# Autodesk Inventor assembly: LearningKitSolarAlt
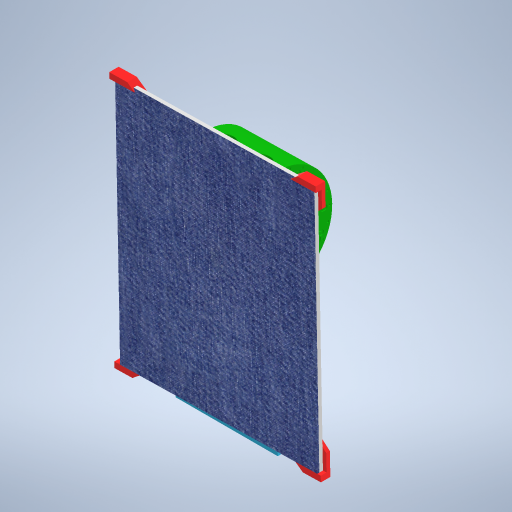
[picture p0: Inventor's stored thumbnail of the model, 512x512]
Saved by Autodesk Inventor 2024.3 (Build 283343000, 343)
## iProperties
Created: 2025-02-03
Part Number: LearningKitSolarAlt
Document SubType Name: Assembly
Designer: Maximilian Hock
Author: Maximilian Hock
## Documents named in this file (6)
- Z:\Dokumente\LearningKit\LearningKitSolar\LearningKitSolar.iam
- Z:\Dokumente\LearningKit\LearningKitSolar\SolarCradle.ipt
- Z:\Dokumente\LearningKit\LearningKitSolar\SolarFoot.ipt
- Z:\Dokumente\LearningKit\LearningKitSolar\SolarScale.ipt
- Z:\Dokumente\LearningKit\LearningKitSolar\SolarPanel.ipt
- Z:\Dokumente\LearningKit\LearningKitSolar\SolarPlugAdapter.ipt
## Components (6 placed, 5 different names)
1. SolarCradle:1 — Planar:1, Starr:1, Starr:2
2. SolarFoot:1 — Passend:1, Passend:3, Drehbar:1, Passend:4
3. SolarScale:1 — Planar:1, Starr:1, Drehbar:1, Zylindrisch:1, Planar:2
4. SolarPanel:1 — Starr:2
5. SolarPlugAdapter:1 — Zylindrisch:1, Planar:2
6. SolarPlugAdapter:2
## Relationships (9: Mate 3, PlanarJoint 2, WeldJoint 2, RevoluteJoint 1, CylindricalJoint 1)
- Passend:1 [Mate]: SolarFoot:1
- Passend:3 [Mate]: SolarFoot:1
- Planar:1: SolarCradle:1 ↔ SolarScale:1
- Starr:1 [WeldJoint]: SolarCradle:1 ↔ SolarScale:1
- Drehbar:1 [RevoluteJoint]: SolarFoot:1 ↔ SolarScale:1
- Starr:2 [WeldJoint]: SolarCradle:1 ↔ SolarPanel:1
- Passend:4 [Mate]: SolarFoot:1
- Zylindrisch:1 [CylindricalJoint]: SolarScale:1 ↔ SolarPlugAdapter:1
- Planar:2: SolarScale:1 ↔ SolarPlugAdapter:1
